# Autodesk Inventor assembly: Blesson Thomas_9005538_Final
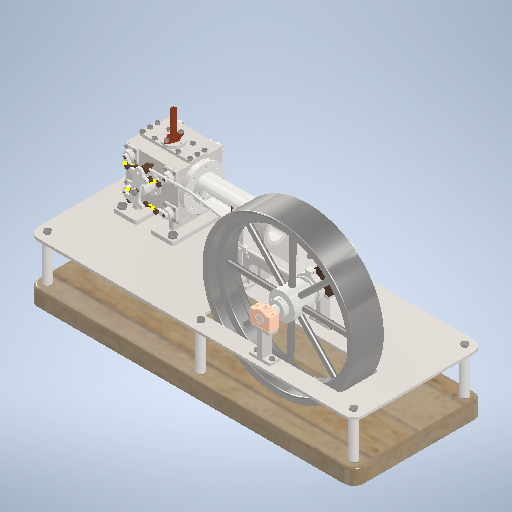
[picture p0: Inventor's stored thumbnail of the model, 512x512]
Saved by Autodesk Inventor 2025.2 (Build 292293000, 293)
## iProperties
Created: 2025-08-11
Part Number: Blesson Thomas_9005538_Final
Document SubType Name: Assembly
Designer: bless
Author: bless
## Documents named in this file (57)
- C:\Users\bless\OneDrive - Conestoga College\Documents\Inventor\pipe and flange\Blesson Thomas_9005538_Final\Blesson Thomas_9005538_Final.iam
- C:\Users\bless\OneDrive - Conestoga College\Documents\Inventor\pipe and flange\Blesson Thomas_9005538_Final\35 - Wooden Base.ipt
- C:\Users\bless\OneDrive - Conestoga College\Documents\Inventor\pipe and flange\Blesson Thomas_9005538_Final\34 - Base Pillar.ipt
- C:\Users\bless\OneDrive - Conestoga College\Documents\Inventor\Content Center Files\R2025\en-US\AS 1237 (2.1)\AS 1237 - 5.ipt
- C:\Users\bless\OneDrive - Conestoga College\Documents\Inventor\pipe and flange\Blesson Thomas_9005538_Final\01 - Base Plate\01 - Base Plate\01 - Base Plate.ipt
- C:\Users\bless\OneDrive - Conestoga College\Documents\Inventor\Content Center Files\R2025\en-US\AS 1110\AS 1110 - M4 x 40.ipt
- C:\Users\bless\OneDrive - Conestoga College\Documents\Inventor\pipe and flange\Blesson Thomas_9005538_Final\03 - Cylinder Foot\03 - Cylinder Foot\03 - Cylinder Foot.ipt
- C:\Users\bless\OneDrive - Conestoga College\Documents\Inventor\Content Center Files\R2025\en-US\AS 1110\AS 1110 - M5 x 12.ipt
- C:\Users\bless\OneDrive - Conestoga College\Documents\Inventor\pipe and flange\Blesson Thomas_9005538_Final\04A - Guide Support 1\04A - Guide Support 1\04A - Guide Support 1.ipt
- C:\Users\bless\OneDrive - Conestoga College\Documents\Inventor\Content Center Files\R2025\en-US\AS 1110\AS 1110 - M2.5 x 8.ipt
- C:\Users\bless\OneDrive - Conestoga College\Documents\Inventor\pipe and flange\Blesson Thomas_9005538_Final\04B - Guide Support 2\04B - Guide Support 2\04B - Guide Support 2.ipt
- C:\Users\bless\OneDrive - Conestoga College\Documents\Inventor\Content Center Files\R2025\en-US\AS 1110\AS 1110 - M2.5 x 12.ipt
- C:\Users\bless\OneDrive - Conestoga College\Documents\Inventor\pipe and flange\Blesson Thomas_9005538_Final\06 - Cylinder\06 - Cylinder\06 - Cylinder.ipt
- C:\Users\bless\OneDrive - Conestoga College\Documents\Inventor\pipe and flange\Blesson Thomas_9005538_Final\09 - Valve Chest Cover Plate\09 - Valve Chest Cover Plate\09 - Valve Chest Cover Plate.ipt
- C:\Users\bless\OneDrive - Conestoga College\Documents\Inventor\Content Center Files\R2025\en-US\AS 1110\AS 1110 - M2.5 x 6.ipt
- C:\Users\bless\OneDrive - Conestoga College\Documents\Inventor\pipe and flange\Blesson Thomas_9005538_Final\36 - Inlet Outlet Steam Pipe.ipt
- C:\Users\bless\OneDrive - Conestoga College\Documents\Inventor\pipe and flange\Blesson Thomas_9005538_Final\12B VALVE BONNET.ipt
- C:\Users\bless\OneDrive - Conestoga College\Documents\Inventor\Content Center Files\R2025\en-US\AS 1110\AS 1110 - M1.6 x 6.ipt
- C:\Users\bless\OneDrive - Conestoga College\Documents\Inventor\pipe and flange\Blesson Thomas_9005538_Final\07 CYLINDER FRONT COVER.ipt
- C:\Users\bless\OneDrive - Conestoga College\Documents\Inventor\pipe and flange\Blesson Thomas_9005538_Final\08 CYLINDER REAR COVER.ipt
- C:\Users\bless\OneDrive - Conestoga College\Documents\Inventor\pipe and flange\Blesson Thomas_9005538_Final\13A FLYWHEEL HUB.ipt
- C:\Users\bless\OneDrive - Conestoga College\Documents\Inventor\pipe and flange\Blesson Thomas_9005538_Final\Flywheel inner ring.ipt
- C:\Users\bless\OneDrive - Conestoga College\Documents\Inventor\pipe and flange\Blesson Thomas_9005538_Final\Flywheel outer rim.ipt
- C:\Users\bless\OneDrive - Conestoga College\Documents\Inventor\pipe and flange\Blesson Thomas_9005538_Final\Flywheel Spoke.ipt
- C:\Users\bless\OneDrive - Conestoga College\Documents\Inventor\pipe and flange\Blesson Thomas_9005538_Final\02 - Outrigger Bearing Pedestal\02 - Outrigger Bearing Pedestal\02 - Outrigger Bearing Pedestal.ipt
- C:\Users\bless\OneDrive - Conestoga College\Documents\Inventor\pipe and flange\Blesson Thomas_9005538_Final\05 Crankbearing.ipt
- C:\Users\bless\OneDrive - Conestoga College\Documents\Inventor\pipe and flange\Blesson Thomas_9005538_Final\02 - Outrigger Bearing Pedestal\05 - Crankshaft Bearing\05 - Crankshaft Bearing.ipt
- C:\Users\bless\OneDrive - Conestoga College\Documents\Inventor\pipe and flange\Blesson Thomas_9005538_Final\Crankshaft.ipt
- C:\Users\bless\OneDrive - Conestoga College\Documents\Inventor\pipe and flange\Blesson Thomas_9005538_Final\28 - Eccentric  Sheav.ipt
- C:\Users\bless\OneDrive - Conestoga College\Documents\Inventor\pipe and flange\Blesson Thomas_9005538_Final\29 - Sheave Strap 2.ipt
- C:\Users\bless\OneDrive - Conestoga College\Documents\Inventor\pipe and flange\Blesson Thomas_9005538_Final\29 - Sheave Strap 1.ipt
- C:\Users\bless\OneDrive - Conestoga College\Documents\Inventor\pipe and flange\Blesson Thomas_9005538_Final\30 - Eccentric Rod 1.ipt
- C:\Users\bless\OneDrive - Conestoga College\Documents\Inventor\pipe and flange\Blesson Thomas_9005538_Final\30 - Eccentric Rod 2.ipt
- C:\Users\bless\OneDrive - Conestoga College\Documents\Inventor\pipe and flange\Blesson Thomas_9005538_Final\31 - Lever.ipt
- C:\Users\bless\OneDrive - Conestoga College\Documents\Inventor\pipe and flange\Blesson Thomas_9005538_Final\32 - Eccentric Disk Rod.ipt
- C:\Users\bless\OneDrive - Conestoga College\Documents\Inventor\pipe and flange\Blesson Thomas_9005538_Final\22 - Valve Disc Hub.ipt
- C:\Users\bless\OneDrive - Conestoga College\Documents\Inventor\pipe and flange\Blesson Thomas_9005538_Final\33 - Eccentric Swivel Screw.ipt
- C:\Users\bless\OneDrive - Conestoga College\Documents\Inventor\pipe and flange\Blesson Thomas_9005538_Final\24 - Valve Disc Spindle.ipt
- C:\Users\bless\OneDrive - Conestoga College\Documents\Inventor\pipe and flange\Blesson Thomas_9005538_Final\23 - Valve Disc.ipt
- C:\Users\bless\OneDrive - Conestoga College\Documents\Inventor\Content Center Files\R2025\en-US\ANSI B18.2.4.2M\ANSI B18.2.4.2M - M3x0.5 - 5.5.ipt
- C:\Users\bless\OneDrive - Conestoga College\Documents\Inventor\pipe and flange\Blesson Thomas_9005538_Final\27 - Valve Level.ipt
- C:\Users\bless\OneDrive - Conestoga College\Documents\Inventor\pipe and flange\Blesson Thomas_9005538_Final\11 CROSSHEAD GUIDE.ipt
- C:\Users\bless\OneDrive - Conestoga College\Documents\Inventor\pipe and flange\Blesson Thomas_9005538_Final\25 - Disc Arm 1.ipt
- C:\Users\bless\OneDrive - Conestoga College\Documents\Inventor\pipe and flange\Blesson Thomas_9005538_Final\25 - Disc Arm 2.ipt
- C:\Users\bless\OneDrive - Conestoga College\Documents\Inventor\pipe and flange\Blesson Thomas_9005538_Final\26B - Valve spindle.ipt
- C:\Users\bless\OneDrive - Conestoga College\Documents\Inventor\pipe and flange\Blesson Thomas_9005538_Final\26A - Valve.ipt
- C:\Users\bless\OneDrive - Conestoga College\Documents\Inventor\pipe and flange\Blesson Thomas_9005538_Final\10a GLAND NUT.ipt
- C:\Users\bless\OneDrive - Conestoga College\Documents\Inventor\pipe and flange\Blesson Thomas_9005538_Final\10B - Gland Nut Seal\10B - Gland Nut Seal\10B - Gland Nut Seal.ipt
- C:\Users\bless\OneDrive - Conestoga College\Documents\Inventor\pipe and flange\Blesson Thomas_9005538_Final\16C - Con Head Crosshead.ipt
- C:\Users\bless\OneDrive - Conestoga College\Documents\Inventor\pipe and flange\Blesson Thomas_9005538_Final\19 - Crosshead.ipt
- C:\Users\bless\OneDrive - Conestoga College\Documents\Inventor\pipe and flange\Blesson Thomas_9005538_Final\18 - Piston Rod.ipt
- C:\Users\bless\OneDrive - Conestoga College\Documents\Inventor\pipe and flange\Blesson Thomas_9005538_Final\21 - Piston Ring.ipt
- C:\Users\bless\OneDrive - Conestoga College\Documents\Inventor\pipe and flange\Blesson Thomas_9005538_Final\20 - Piston.ipt
- C:\Users\bless\OneDrive - Conestoga College\Documents\Inventor\pipe and flange\Blesson Thomas_9005538_Final\16B2 - Con Head Big End.ipt
- C:\Users\bless\OneDrive - Conestoga College\Documents\Inventor\pipe and flange\Blesson Thomas_9005538_Final\16A - Con Rod.ipt
- C:\Users\bless\OneDrive - Conestoga College\Documents\Inventor\pipe and flange\Blesson Thomas_9005538_Final\17B - Crosshead Pin2.ipt
- C:\Users\bless\OneDrive - Conestoga College\Documents\Inventor\pipe and flange\Blesson Thomas_9005538_Final\Crankpin.ipt
## Components (176 placed, 56 different names)
1. 35 - Wooden Base:1 — Insert:1, Insert:2, Insert:3, Insert:4, Insert:5, Insert:6
2. 34 - Base Pillar:1 — Rigid:2
3. 34 - Base Pillar:2 — Rigid:4
4. 34 - Base Pillar:3 — Rigid:6, Cylindrical:1
5. 34 - Base Pillar:4 — Rigid:1, Rigid:7
6. 34 - Base Pillar:5 — Rigid:3
7. 34 - Base Pillar:6 — Rigid:5
8. AS 1237 (2.1) 5:1 — Insert:1, Rigid:1
9. AS 1237 (2.1) 5:2 — Insert:2, Rigid:2
10. AS 1237 (2.1) 5:3 — Insert:3, Rigid:4
11. AS 1237 (2.1) 5:4 — Insert:4, Rigid:5
12. AS 1237 (2.1) 5:5 — Insert:5, Rigid:6
13. AS 1237 (2.1) 5:6 — Insert:6, Rigid:3
14. 01 - Base Plate:1 — Rigid:7, Insert:7, Insert:8, Insert:9, Insert:10, Insert:11, Insert:12, Rotational:1, Cylindrical:2, Rotational:2, Cylindrical:3, Rotational:3, Cylindrical:4, Cylindrical:5, Cylindrical:6, Cylindrical:14, Cylindrical:44, Mate:27, Cylindrical:49
15. AS 1110 - Metric M4 x 40:1 — Insert:7
16. AS 1110 - Metric M4 x 40:2 — Insert:8
17. AS 1110 - Metric M4 x 40:3 — Insert:9
18. AS 1110 - Metric M4 x 40:4 — Insert:10
19. AS 1110 - Metric M4 x 40:5 — Insert:11
20. AS 1110 - Metric M4 x 40:6 — Insert:12, Cylindrical:1
21. 03 - Cylinder Foot:1 — Rotational:1, Insert:13, Insert:14
22. 03 - Cylinder Foot:2 — Rotational:2, Insert:15, Insert:16, Angle:1, Mate:7
23. AS 1110 - Metric M5 x 12:1 — Insert:13
24. AS 1110 - Metric M5 x 12:2 — Insert:14, Cylindrical:2
25. AS 1110 - Metric M5 x 12:3 — Insert:15
26. AS 1110 - Metric M5 x 12:4 — Insert:16, Cylindrical:3
27. 04A - Guide Support 1:1 — Insert:17, Insert:18, Rotational:3, Mate:1, Cylindrical:70
28. AS 1110 - Metric M2.5 x 8:1 — Insert:17
29. AS 1110 - Metric M2.5 x 8:2 — Insert:18, Cylindrical:4
30. 04B - Guide Support 2:1 — Mate:1, Insert:19, Insert:20, Cylindrical:45, Mate:28, Flush:3, Cylindrical:60
31. AS 1110 - Metric M2.5 x 12:1 — Insert:19, Cylindrical:5
32. AS 1110 - Metric M2.5 x 12:2 — Insert:20, Cylindrical:6
33. 06 - Cylinder:1 — Cylindrical:7, Mate:2, Cylindrical:13, Cylindrical:15, Cylindrical:16, Cylindrical:17, Mate:6, Mate:7, Cylindrical:18, Cylindrical:19, Mate:8, Cylindrical:20, Cylindrical:21, Mate:9, Cylindrical:22, Cylindrical:23, Mate:10, Cylindrical:24, Cylindrical:25, Mate:11, Cylindrical:26, Cylindrical:27, Mate:12, Mate:13, Cylindrical:28, Cylindrical:29, Mate:14, Cylindrical:30, Cylindrical:31, Cylindrical:32, Cylindrical:33, Mate:16, Mate:17, Cylindrical:61, Mate:40
34. 09 - Valve Chest Cover Plate:1 — Insert:21, Insert:22, Insert:23, Insert:24, Insert:25, Insert:26, Insert:27, Insert:28, Insert:29, Insert:30, Mate:2, Cylindrical:11, Cylindrical:12, Mate:5
35. 09 - Valve Chest Cover Plate:2 — Insert:32, Insert:33, Insert:34, Insert:35, Insert:36, Insert:37, Insert:38, Insert:39, Insert:40, Cylindrical:9, Cylindrical:10, Mate:4, Mate:6, Angle:1
36. AS 1110 - Metric M2.5 x 6:1 — Insert:21
37. AS 1110 - Metric M2.5 x 6:2 — Insert:22, Cylindrical:7
38. AS 1110 - Metric M2.5 x 6:3 — Insert:23
39. AS 1110 - Metric M2.5 x 6:4 — Insert:24
40. AS 1110 - Metric M2.5 x 6:5 — Insert:25
41. AS 1110 - Metric M2.5 x 6:6 — Insert:26, Cylindrical:13
42. AS 1110 - Metric M2.5 x 6:7 — Insert:27
43. AS 1110 - Metric M2.5 x 6:8 — Insert:28
44. AS 1110 - Metric M2.5 x 6:9 — Insert:29
45. AS 1110 - Metric M2.5 x 6:10 — Insert:30
46. AS 1110 - Metric M2.5 x 6:12 — Insert:32
47. AS 1110 - Metric M2.5 x 6:13 — Insert:33, Cylindrical:17
48. AS 1110 - Metric M2.5 x 6:14 — Insert:34
49. AS 1110 - Metric M2.5 x 6:15 — Insert:35
50. AS 1110 - Metric M2.5 x 6:16 — Insert:36, Cylindrical:15
51. AS 1110 - Metric M2.5 x 6:17 — Insert:37
52. AS 1110 - Metric M2.5 x 6:18 — Insert:38
53. AS 1110 - Metric M2.5 x 6:19 — Insert:39, Cylindrical:16
54. AS 1110 - Metric M2.5 x 6:20 — Insert:40
55. 36 - Inlet Outlet Steam Pipe:1 — Insert:43, Insert:44, Mate:5
56. 36 - Inlet Outlet Steam Pipe:2 — Insert:41, Insert:42, Mate:4, Cylindrical:14
57. AS 1110 - Metric M2.5 x 6:21 — Insert:41, Cylindrical:9
58. AS 1110 - Metric M2.5 x 6:22 — Insert:42, Cylindrical:10
59. AS 1110 - Metric M2.5 x 6:23 — Insert:43, Cylindrical:11
60. AS 1110 - Metric M2.5 x 6:24 — Insert:44, Cylindrical:12
61. 12B VALVE BONNET:1 — Insert:61, Insert:62, Insert:63, Insert:64, Mate:9, Cylindrical:66, Mate:46
62. 12B VALVE BONNET:2 — Insert:65, Insert:66, Insert:67, Insert:68, Mate:11, Cylindrical:67, Mate:47
63. 12B VALVE BONNET:3 — Insert:73, Insert:74, Insert:75, Insert:76, Mate:8, Cylindrical:65, Mate:45
64. 12B VALVE BONNET:4 — Insert:69, Insert:70, Insert:71, Insert:72, Mate:10, Cylindrical:68, Mate:48
65. 12B VALVE BONNET:5 — Insert:57, Insert:58, Insert:59, Insert:60, Mate:13, Cylindrical:28
66. 12B VALVE BONNET:6 — Insert:53, Insert:54, Insert:55, Insert:56, Flush:1
67. 12B VALVE BONNET:7 — Insert:45, Insert:46, Insert:47, Insert:48, Cylindrical:29, Mate:14, Flush:1
68. 12B VALVE BONNET:8 — Insert:49, Insert:50, Insert:51, Insert:52, Mate:12
69. AS 1110 - Metric M1.6 x 6:1 — Insert:45
70. AS 1110 - Metric M1.6 x 6:2 — Insert:46
71. AS 1110 - Metric M1.6 x 6:3 — Insert:47
72. AS 1110 - Metric M1.6 x 6:4 — Insert:48, Cylindrical:30
73. AS 1110 - Metric M1.6 x 6:5 — Insert:49, Cylindrical:27
74. AS 1110 - Metric M1.6 x 6:6 — Insert:50
75. AS 1110 - Metric M1.6 x 6:7 — Insert:51, Cylindrical:26
76. AS 1110 - Metric M1.6 x 6:8 — Insert:52
77. AS 1110 - Metric M1.6 x 6:9 — Insert:53, Cylindrical:32
78. AS 1110 - Metric M1.6 x 6:10 — Insert:54, Cylindrical:33
79. AS 1110 - Metric M1.6 x 6:11 — Insert:55
80. AS 1110 - Metric M1.6 x 6:12 — Insert:56
81. AS 1110 - Metric M1.6 x 6:13 — Insert:57
82. AS 1110 - Metric M1.6 x 6:14 — Insert:58
83. AS 1110 - Metric M1.6 x 6:15 — Insert:59
84. AS 1110 - Metric M1.6 x 6:16 — Insert:60, Cylindrical:31
85. AS 1110 - Metric M1.6 x 6:17 — Insert:61
86. AS 1110 - Metric M1.6 x 6:18 — Insert:62, Cylindrical:21
87. AS 1110 - Metric M1.6 x 6:19 — Insert:63, Cylindrical:20
88. AS 1110 - Metric M1.6 x 6:20 — Insert:64
89. AS 1110 - Metric M1.6 x 6:21 — Insert:65
90. AS 1110 - Metric M1.6 x 6:22 — Insert:66, Cylindrical:25
91. AS 1110 - Metric M1.6 x 6:23 — Insert:67, Cylindrical:24
92. AS 1110 - Metric M1.6 x 6:24 — Insert:68
93. AS 1110 - Metric M1.6 x 6:25 — Insert:69, Cylindrical:23
94. AS 1110 - Metric M1.6 x 6:26 — Insert:70, Cylindrical:22
95. AS 1110 - Metric M1.6 x 6:27 — Insert:71
96. AS 1110 - Metric M1.6 x 6:28 — Insert:72
97. AS 1110 - Metric M1.6 x 6:29 — Insert:73, Cylindrical:18
98. AS 1110 - Metric M1.6 x 6:30 — Insert:74, Cylindrical:19
99. AS 1110 - Metric M1.6 x 6:31 — Insert:75
100. AS 1110 - Metric M1.6 x 6:32 — Insert:76
101. 07 CYLINDER FRONT COVER:1 — Insert:77, Insert:78, Insert:79, Insert:80, Insert:81, Insert:82, Insert:83, Insert:84, Mate:16
102. AS 1110 - Metric M2.5 x 6:25 — Insert:77
103. AS 1110 - Metric M2.5 x 6:26 — Insert:78
104. AS 1110 - Metric M2.5 x 6:27 — Insert:79
105. AS 1110 - Metric M2.5 x 6:28 — Insert:80
106. AS 1110 - Metric M2.5 x 6:29 — Insert:81
107. AS 1110 - Metric M2.5 x 6:30 — Insert:82
108. AS 1110 - Metric M2.5 x 6:31 — Insert:83
109. AS 1110 - Metric M2.5 x 6:32 — Insert:84
110. 08 CYLINDER REAR COVER:1 — Mate:17, Cylindrical:69, Mate:71, Mate:74
111. 13A FLYWHEEL HUB:1 — Cylindrical:34, Cylindrical:35, Cylindrical:36, Cylindrical:37, Mate:15, Mate:18, Mate:19, Mate:20, Cylindrical:38, Mate:21, Cylindrical:39, Cylindrical:40, Cylindrical:41, Mate:22, Mate:23, Mate:24, Cylindrical:51, Cylindrical:52, Cylindrical:54
112. Flywheel inner ring:1 — Cylindrical:42, Cylindrical:43, Mate:25, Insert:95
113. Flywheel outer rim:1 — Mate:25, Insert:95
114. Flywheel Spoke:1 — Cylindrical:34, Mate:18
115. Flywheel Spoke:2 — Cylindrical:39, Mate:24
116. Flywheel Spoke:3 — Cylindrical:38, Mate:21
117. Flywheel Spoke:4 — Cylindrical:35, Mate:15
118. Flywheel Spoke:5 — Cylindrical:40, Mate:22, Cylindrical:42
119. Flywheel Spoke:6 — Cylindrical:41, Mate:23, Cylindrical:43
120. Flywheel Spoke:7 — Cylindrical:37, Mate:20
121. Flywheel Spoke:8 — Cylindrical:36, Mate:19
122. 02 - Outrigger Bearing Pedestal:2 — Insert:93, Insert:94, Mate:26, Mate:27, Flush:2, Mate:29, Flush:4
123. AS 1110 - Metric M2.5 x 6:41 — Insert:93, Cylindrical:44
124. AS 1110 - Metric M2.5 x 6:42 — Insert:94, Cylindrical:49
125. 05 Crankbearing:1 — Cylindrical:45, Mate:28, Flush:3
126. 05 - Crankshaft Bearing:1 — Mate:26, Flush:2, Mate:29, Flush:4, Flush:5, Cylindrical:50, Cylindrical:51
127. Crankshaft:1 — Flush:5, Cylindrical:50, Cylindrical:52, Mate:31, Cylindrical:96
128. 28 - Eccentric  Sheav:1 — Mate:31, Mate:33, Flush:7, Cylindrical:54, Mate:35
129. 29 - Sheave Strap 2:1 — Cylindrical:53, Mate:32, Mate:34, Flush:6, Flush:7
130. 29 - Sheave Strap 1:1 — Cylindrical:53, Mate:32, Mate:33, Mate:34, Flush:6, Cylindrical:55
131. 30 - Eccentric Rod 1:1 — Cylindrical:55, Mate:35, Cylindrical:56, Mate:36
132. 30 - Eccentric Rod 2:1 — Cylindrical:56, Mate:36, Cylindrical:57, Mate:37
133. 31 - Lever:1 — Cylindrical:57, Mate:37, Cylindrical:59, Mate:39, Cylindrical:60
134. 32 - Eccentric Disk Rod:1 — Cylindrical:58, Mate:38, Cylindrical:62
135. 30 - Eccentric Rod 2:2 — Cylindrical:58, Mate:38, Cylindrical:59, Mate:39
136. 22 - Valve Disc Hub:2 — Cylindrical:61, Mate:40, Cylindrical:63, Flush:8
137. 33 - Eccentric Swivel Screw:1 — Cylindrical:62, Cylindrical:64
138. 24 - Valve Disc Spindle:1 — Cylindrical:63, Flush:8, Mate:41, Mate:42, Flush:9, Mate:43, Mate:44
139. 23 - Valve Disc:1 — Mate:41, Mate:42, Cylindrical:64, Flush:9, Cylindrical:75, Cylindrical:76, Cylindrical:77, Cylindrical:78
140. ANSI B18.2.4.2M M3x0.5:1 — Mate:43, Mate:44
141. 27 - Valve Level:1 — Cylindrical:65, Mate:45, Cylindrical:71, Mate:58, Cylindrical:84
142. 27 - Valve Level:2 — Cylindrical:66, Mate:46, Cylindrical:72, Mate:59, Cylindrical:85
143. 27 - Valve Level:3 — Cylindrical:67, Mate:47, Cylindrical:74, Mate:60, Cylindrical:86
144. 27 - Valve Level:4 — Cylindrical:68, Mate:48, Cylindrical:73, Mate:61, Cylindrical:83
145. 11 CROSSHEAD GUIDE:1 — Cylindrical:69, Cylindrical:70, Cylindrical:91, Mate:74
146. 25 - Disc Arm 1:1 — Mate:56, Cylindrical:76
147. 25 - Disc Arm 1:2 — Mate:54, Cylindrical:73, Mate:61
148. 25 - Disc Arm 1:3 — Mate:52, Cylindrical:78
149. 25 - Disc Arm 1:4 — Mate:49, Mate:50, Mate:58, Cylindrical:75
150. 25 - Disc Arm 1:5 — Mate:51, Cylindrical:71
151. 25 - Disc Arm 1:6 — Mate:53, Cylindrical:74, Mate:60
152. 25 - Disc Arm 1:7 — Mate:55, Cylindrical:77
153. 25 - Disc Arm 1:8 — Mate:57, Cylindrical:72, Mate:59
154. 25 - Disc Arm 2:1 — Mate:49, Mate:50, Mate:51
155. 25 - Disc Arm 2:2 — Mate:52, Mate:53
156. 25 - Disc Arm 2:3 — Mate:54, Mate:55
157. 25 - Disc Arm 2:4 — Mate:56, Mate:57
158. 26B - Valve spindle:1 — Mate:62, Cylindrical:79, Mate:63, Cylindrical:83
159. 26A - Valve:1 — Mate:62, Cylindrical:79, Mate:63
160. 26B - Valve spindle:2 — Cylindrical:84
161. 26A - Valve:2
162. 26B - Valve spindle:3 — Cylindrical:85
163. 26A - Valve:3
164. 26B - Valve spindle:4 — Cylindrical:86
165. 26A - Valve:4
166. 10a GLAND NUT:1 — Cylindrical:87, Mate:70
167. 10B - Gland Nut Seal:1 — Cylindrical:87, Mate:70, Mate:71
168. 16C - Con Head Crosshead:1 — Mate:76, Cylindrical:92, Mate:77, Cylindrical:94, Mate:78
169. 19 - Crosshead:1 — Cylindrical:88, Mate:72, Cylindrical:93, Mate:78
170. 18 - Piston Rod:1 — Cylindrical:88, Mate:72, Cylindrical:90, Flush:10
171. 21 - Piston Ring:1 — Cylindrical:89, Mate:73
172. 20 - Piston:1 — Cylindrical:89, Mate:73, Cylindrical:90, Flush:10, Cylindrical:91
173. 16B2 - Con Head Big End:1 — Mate:75, Cylindrical:95, Cylindrical:96, Cylindrical:97
174. 16A - Con Rod:1 — Mate:75, Mate:76, Cylindrical:94, Cylindrical:95
175. 17B - Crosshead Pin2:1 — Cylindrical:92, Mate:77, Cylindrical:93
176. Crankpin:1 — Cylindrical:97
## Relationships (276: CylindricalJoint 93, Insert 86, Mate 76, Flush 10, WeldJoint 7, RevoluteJoint 3, Angle 1)
- Insert:1: 35 - Wooden Base:1 ↔ AS 1237 (2.1) 5:1
- Insert:2: 35 - Wooden Base:1 ↔ AS 1237 (2.1) 5:2
- Insert:3: 35 - Wooden Base:1 ↔ AS 1237 (2.1) 5:3
- Insert:4: 35 - Wooden Base:1 ↔ AS 1237 (2.1) 5:4
- Insert:5: 35 - Wooden Base:1 ↔ AS 1237 (2.1) 5:5
- Insert:6: 35 - Wooden Base:1 ↔ AS 1237 (2.1) 5:6
- Rigid:1 [WeldJoint]: 34 - Base Pillar:4 ↔ AS 1237 (2.1) 5:1
- Rigid:2 [WeldJoint]: 34 - Base Pillar:1 ↔ AS 1237 (2.1) 5:2
- Rigid:3 [WeldJoint]: 34 - Base Pillar:5 ↔ AS 1237 (2.1) 5:6
- Rigid:4 [WeldJoint]: 34 - Base Pillar:2 ↔ AS 1237 (2.1) 5:3
- Rigid:5 [WeldJoint]: 34 - Base Pillar:6 ↔ AS 1237 (2.1) 5:4
- Rigid:6 [WeldJoint]: 34 - Base Pillar:3 ↔ AS 1237 (2.1) 5:5
- Rigid:7 [WeldJoint]: 34 - Base Pillar:4 ↔ 01 - Base Plate:1
- Insert:7: 01 - Base Plate:1 ↔ AS 1110 - Metric M4 x 40:1
- Insert:8: 01 - Base Plate:1 ↔ AS 1110 - Metric M4 x 40:2
- Insert:9: 01 - Base Plate:1 ↔ AS 1110 - Metric M4 x 40:3
- Insert:10: 01 - Base Plate:1 ↔ AS 1110 - Metric M4 x 40:4
- Insert:11: 01 - Base Plate:1 ↔ AS 1110 - Metric M4 x 40:5
- Insert:12: 01 - Base Plate:1 ↔ AS 1110 - Metric M4 x 40:6
- Rotational:1 [RevoluteJoint]: 01 - Base Plate:1 ↔ 03 - Cylinder Foot:1
- Cylindrical:1: 34 - Base Pillar:3 ↔ AS 1110 - Metric M4 x 40:6
- Insert:13: 03 - Cylinder Foot:1 ↔ AS 1110 - Metric M5 x 12:1
- Insert:14: 03 - Cylinder Foot:1 ↔ AS 1110 - Metric M5 x 12:2
- Cylindrical:2: 01 - Base Plate:1 ↔ AS 1110 - Metric M5 x 12:2
- Rotational:2 [RevoluteJoint]: 01 - Base Plate:1 ↔ 03 - Cylinder Foot:2
- Insert:15: 03 - Cylinder Foot:2 ↔ AS 1110 - Metric M5 x 12:3
- Insert:16: 03 - Cylinder Foot:2 ↔ AS 1110 - Metric M5 x 12:4
- Cylindrical:3: 01 - Base Plate:1 ↔ AS 1110 - Metric M5 x 12:4
- Insert:17: 04A - Guide Support 1:1 ↔ AS 1110 - Metric M2.5 x 8:1
- Insert:18: 04A - Guide Support 1:1 ↔ AS 1110 - Metric M2.5 x 8:2
- Rotational:3 [RevoluteJoint]: 01 - Base Plate:1 ↔ 04A - Guide Support 1:1
- Cylindrical:4: 01 - Base Plate:1 ↔ AS 1110 - Metric M2.5 x 8:2
- Mate:1: 04A - Guide Support 1:1 ↔ 04B - Guide Support 2:1
- Insert:19: 04B - Guide Support 2:1 ↔ AS 1110 - Metric M2.5 x 12:1
- Insert:20: 04B - Guide Support 2:1 ↔ AS 1110 - Metric M2.5 x 12:2
- Cylindrical:5: 01 - Base Plate:1 ↔ AS 1110 - Metric M2.5 x 12:1
- Cylindrical:6: 01 - Base Plate:1 ↔ AS 1110 - Metric M2.5 x 12:2
- Insert:21: 09 - Valve Chest Cover Plate:1 ↔ AS 1110 - Metric M2.5 x 6:1
- Insert:22: 09 - Valve Chest Cover Plate:1 ↔ AS 1110 - Metric M2.5 x 6:2
- Insert:23: 09 - Valve Chest Cover Plate:1 ↔ AS 1110 - Metric M2.5 x 6:3
- Insert:24: 09 - Valve Chest Cover Plate:1 ↔ AS 1110 - Metric M2.5 x 6:4
- Insert:25: 09 - Valve Chest Cover Plate:1 ↔ AS 1110 - Metric M2.5 x 6:5
- Insert:26: 09 - Valve Chest Cover Plate:1 ↔ AS 1110 - Metric M2.5 x 6:6
- Insert:27: 09 - Valve Chest Cover Plate:1 ↔ AS 1110 - Metric M2.5 x 6:7
- Insert:28: 09 - Valve Chest Cover Plate:1 ↔ AS 1110 - Metric M2.5 x 6:8
- Insert:29: 09 - Valve Chest Cover Plate:1 ↔ AS 1110 - Metric M2.5 x 6:9
- Insert:30: 09 - Valve Chest Cover Plate:1 ↔ AS 1110 - Metric M2.5 x 6:10
- Cylindrical:7: 06 - Cylinder:1 ↔ AS 1110 - Metric M2.5 x 6:2
- Mate:2: 06 - Cylinder:1 ↔ 09 - Valve Chest Cover Plate:1
- Insert:32: 09 - Valve Chest Cover Plate:2 ↔ AS 1110 - Metric M2.5 x 6:12
- Insert:33: 09 - Valve Chest Cover Plate:2 ↔ AS 1110 - Metric M2.5 x 6:13
- Insert:34: 09 - Valve Chest Cover Plate:2 ↔ AS 1110 - Metric M2.5 x 6:14
- Insert:35: 09 - Valve Chest Cover Plate:2 ↔ AS 1110 - Metric M2.5 x 6:15
- Insert:36: 09 - Valve Chest Cover Plate:2 ↔ AS 1110 - Metric M2.5 x 6:16
- Insert:37: 09 - Valve Chest Cover Plate:2 ↔ AS 1110 - Metric M2.5 x 6:17
- Insert:38: 09 - Valve Chest Cover Plate:2 ↔ AS 1110 - Metric M2.5 x 6:18
- Insert:39: 09 - Valve Chest Cover Plate:2 ↔ AS 1110 - Metric M2.5 x 6:19
- Insert:40: 09 - Valve Chest Cover Plate:2 ↔ AS 1110 - Metric M2.5 x 6:20
- Insert:41: 36 - Inlet Outlet Steam Pipe:2 ↔ AS 1110 - Metric M2.5 x 6:21
- Insert:42: 36 - Inlet Outlet Steam Pipe:2 ↔ AS 1110 - Metric M2.5 x 6:22
- Insert:43: 36 - Inlet Outlet Steam Pipe:1 ↔ AS 1110 - Metric M2.5 x 6:23
- Insert:44: 36 - Inlet Outlet Steam Pipe:1 ↔ AS 1110 - Metric M2.5 x 6:24
- Cylindrical:9: 09 - Valve Chest Cover Plate:2 ↔ AS 1110 - Metric M2.5 x 6:21
- Cylindrical:10: 09 - Valve Chest Cover Plate:2 ↔ AS 1110 - Metric M2.5 x 6:22
- Mate:4: 09 - Valve Chest Cover Plate:2 ↔ 36 - Inlet Outlet Steam Pipe:2
- Cylindrical:11: 09 - Valve Chest Cover Plate:1 ↔ AS 1110 - Metric M2.5 x 6:23
- Cylindrical:12: 09 - Valve Chest Cover Plate:1 ↔ AS 1110 - Metric M2.5 x 6:24
- Mate:5: 09 - Valve Chest Cover Plate:1 ↔ 36 - Inlet Outlet Steam Pipe:1
- Cylindrical:13: 06 - Cylinder:1 ↔ AS 1110 - Metric M2.5 x 6:6
- Cylindrical:14: 01 - Base Plate:1 ↔ 36 - Inlet Outlet Steam Pipe:2
- Cylindrical:15: 06 - Cylinder:1 ↔ AS 1110 - Metric M2.5 x 6:16
- Cylindrical:16: 06 - Cylinder:1 ↔ AS 1110 - Metric M2.5 x 6:19
- Cylindrical:17: 06 - Cylinder:1 ↔ AS 1110 - Metric M2.5 x 6:13
- Mate:6: 06 - Cylinder:1 ↔ 09 - Valve Chest Cover Plate:2
- Angle:1 (0 deg): 03 - Cylinder Foot:2 ↔ 09 - Valve Chest Cover Plate:2
- Mate:7: 03 - Cylinder Foot:2 ↔ 06 - Cylinder:1
- Insert:45: 12B VALVE BONNET:7 ↔ AS 1110 - Metric M1.6 x 6:1
- Insert:46: 12B VALVE BONNET:7 ↔ AS 1110 - Metric M1.6 x 6:2
- Insert:47: 12B VALVE BONNET:7 ↔ AS 1110 - Metric M1.6 x 6:3
- Insert:48: 12B VALVE BONNET:7 ↔ AS 1110 - Metric M1.6 x 6:4
- Insert:49: 12B VALVE BONNET:8 ↔ AS 1110 - Metric M1.6 x 6:5
- Insert:50: 12B VALVE BONNET:8 ↔ AS 1110 - Metric M1.6 x 6:6
- Insert:51: 12B VALVE BONNET:8 ↔ AS 1110 - Metric M1.6 x 6:7
- Insert:52: 12B VALVE BONNET:8 ↔ AS 1110 - Metric M1.6 x 6:8
- Insert:53: 12B VALVE BONNET:6 ↔ AS 1110 - Metric M1.6 x 6:9
- Insert:54: 12B VALVE BONNET:6 ↔ AS 1110 - Metric M1.6 x 6:10
- Insert:55: 12B VALVE BONNET:6 ↔ AS 1110 - Metric M1.6 x 6:11
- Insert:56: 12B VALVE BONNET:6 ↔ AS 1110 - Metric M1.6 x 6:12
- Insert:57: 12B VALVE BONNET:5 ↔ AS 1110 - Metric M1.6 x 6:13
- Insert:58: 12B VALVE BONNET:5 ↔ AS 1110 - Metric M1.6 x 6:14
- Insert:59: 12B VALVE BONNET:5 ↔ AS 1110 - Metric M1.6 x 6:15
- Insert:60: 12B VALVE BONNET:5 ↔ AS 1110 - Metric M1.6 x 6:16
- Insert:61: 12B VALVE BONNET:1 ↔ AS 1110 - Metric M1.6 x 6:17
- Insert:62: 12B VALVE BONNET:1 ↔ AS 1110 - Metric M1.6 x 6:18
- Insert:63: 12B VALVE BONNET:1 ↔ AS 1110 - Metric M1.6 x 6:19
- Insert:64: 12B VALVE BONNET:1 ↔ AS 1110 - Metric M1.6 x 6:20
- Insert:65: 12B VALVE BONNET:2 ↔ AS 1110 - Metric M1.6 x 6:21
- Insert:66: 12B VALVE BONNET:2 ↔ AS 1110 - Metric M1.6 x 6:22
- Insert:67: 12B VALVE BONNET:2 ↔ AS 1110 - Metric M1.6 x 6:23
- Insert:68: 12B VALVE BONNET:2 ↔ AS 1110 - Metric M1.6 x 6:24
- Insert:69: 12B VALVE BONNET:4 ↔ AS 1110 - Metric M1.6 x 6:25
- Insert:70: 12B VALVE BONNET:4 ↔ AS 1110 - Metric M1.6 x 6:26
- Insert:71: 12B VALVE BONNET:4 ↔ AS 1110 - Metric M1.6 x 6:27
- Insert:72: 12B VALVE BONNET:4 ↔ AS 1110 - Metric M1.6 x 6:28
- Insert:73: 12B VALVE BONNET:3 ↔ AS 1110 - Metric M1.6 x 6:29
- Insert:74: 12B VALVE BONNET:3 ↔ AS 1110 - Metric M1.6 x 6:30
- Insert:75: 12B VALVE BONNET:3 ↔ AS 1110 - Metric M1.6 x 6:31
- Insert:76: 12B VALVE BONNET:3 ↔ AS 1110 - Metric M1.6 x 6:32
- Cylindrical:18: 06 - Cylinder:1 ↔ AS 1110 - Metric M1.6 x 6:29
- Cylindrical:19: 06 - Cylinder:1 ↔ AS 1110 - Metric M1.6 x 6:30
- Mate:8: 06 - Cylinder:1 ↔ 12B VALVE BONNET:3
- Cylindrical:20: 06 - Cylinder:1 ↔ AS 1110 - Metric M1.6 x 6:19
- Cylindrical:21: 06 - Cylinder:1 ↔ AS 1110 - Metric M1.6 x 6:18
- Mate:9: 06 - Cylinder:1 ↔ 12B VALVE BONNET:1
- Cylindrical:22: 06 - Cylinder:1 ↔ AS 1110 - Metric M1.6 x 6:26
- Cylindrical:23: 06 - Cylinder:1 ↔ AS 1110 - Metric M1.6 x 6:25
- Mate:10: 06 - Cylinder:1 ↔ 12B VALVE BONNET:4
- Cylindrical:24: 06 - Cylinder:1 ↔ AS 1110 - Metric M1.6 x 6:23
- Cylindrical:25: 06 - Cylinder:1 ↔ AS 1110 - Metric M1.6 x 6:22
- Mate:11: 06 - Cylinder:1 ↔ 12B VALVE BONNET:2
- Cylindrical:26: 06 - Cylinder:1 ↔ AS 1110 - Metric M1.6 x 6:7
- Cylindrical:27: 06 - Cylinder:1 ↔ AS 1110 - Metric M1.6 x 6:5
- Mate:12: 06 - Cylinder:1 ↔ 12B VALVE BONNET:8
- Mate:13: 06 - Cylinder:1 ↔ 12B VALVE BONNET:5
- Cylindrical:28: 06 - Cylinder:1 ↔ 12B VALVE BONNET:5
- Cylindrical:29: 06 - Cylinder:1 ↔ 12B VALVE BONNET:7
- Mate:14: 06 - Cylinder:1 ↔ 12B VALVE BONNET:7
- Cylindrical:30: 06 - Cylinder:1 ↔ AS 1110 - Metric M1.6 x 6:4
- Cylindrical:31: 06 - Cylinder:1 ↔ AS 1110 - Metric M1.6 x 6:16
- Cylindrical:32: 06 - Cylinder:1 ↔ AS 1110 - Metric M1.6 x 6:9
- Cylindrical:33: 06 - Cylinder:1 ↔ AS 1110 - Metric M1.6 x 6:10
- Flush:1: 12B VALVE BONNET:6 ↔ 12B VALVE BONNET:7
- Insert:77: 07 CYLINDER FRONT COVER:1 ↔ AS 1110 - Metric M2.5 x 6:25
- Insert:78: 07 CYLINDER FRONT COVER:1 ↔ AS 1110 - Metric M2.5 x 6:26
- Insert:79: 07 CYLINDER FRONT COVER:1 ↔ AS 1110 - Metric M2.5 x 6:27
- Insert:80: 07 CYLINDER FRONT COVER:1 ↔ AS 1110 - Metric M2.5 x 6:28
- Insert:81: 07 CYLINDER FRONT COVER:1 ↔ AS 1110 - Metric M2.5 x 6:29
- Insert:82: 07 CYLINDER FRONT COVER:1 ↔ AS 1110 - Metric M2.5 x 6:30
- Insert:83: 07 CYLINDER FRONT COVER:1 ↔ AS 1110 - Metric M2.5 x 6:31
- Insert:84: 07 CYLINDER FRONT COVER:1 ↔ AS 1110 - Metric M2.5 x 6:32
- Cylindrical:34: 13A FLYWHEEL HUB:1 ↔ Flywheel Spoke:1
- Cylindrical:35: 13A FLYWHEEL HUB:1 ↔ Flywheel Spoke:4
- Cylindrical:36: 13A FLYWHEEL HUB:1 ↔ Flywheel Spoke:8
- Cylindrical:37: 13A FLYWHEEL HUB:1 ↔ Flywheel Spoke:7
- Mate:15: 13A FLYWHEEL HUB:1 ↔ Flywheel Spoke:4
- Mate:16: 06 - Cylinder:1 ↔ 07 CYLINDER FRONT COVER:1
- Mate:17: 06 - Cylinder:1 ↔ 08 CYLINDER REAR COVER:1
- Mate:18: 13A FLYWHEEL HUB:1 ↔ Flywheel Spoke:1
- Mate:19: 13A FLYWHEEL HUB:1 ↔ Flywheel Spoke:8
- Mate:20: 13A FLYWHEEL HUB:1 ↔ Flywheel Spoke:7
- Cylindrical:38: 13A FLYWHEEL HUB:1 ↔ Flywheel Spoke:3
- Mate:21: 13A FLYWHEEL HUB:1 ↔ Flywheel Spoke:3
- Cylindrical:39: 13A FLYWHEEL HUB:1 ↔ Flywheel Spoke:2
- Cylindrical:40: 13A FLYWHEEL HUB:1 ↔ Flywheel Spoke:5
- Cylindrical:41: 13A FLYWHEEL HUB:1 ↔ Flywheel Spoke:6
- Mate:22: 13A FLYWHEEL HUB:1 ↔ Flywheel Spoke:5
- Mate:23: 13A FLYWHEEL HUB:1 ↔ Flywheel Spoke:6
- Mate:24: 13A FLYWHEEL HUB:1 ↔ Flywheel Spoke:2
- Cylindrical:42: Flywheel inner ring:1 ↔ Flywheel Spoke:5
- Cylindrical:43: Flywheel inner ring:1 ↔ Flywheel Spoke:6
- Mate:25: Flywheel inner ring:1 ↔ Flywheel outer rim:1
- Insert:93: 02 - Outrigger Bearing Pedestal:2 ↔ AS 1110 - Metric M2.5 x 6:41
- Insert:94: 02 - Outrigger Bearing Pedestal:2 ↔ AS 1110 - Metric M2.5 x 6:42
- Cylindrical:44: 01 - Base Plate:1 ↔ AS 1110 - Metric M2.5 x 6:41
- Cylindrical:45: 04B - Guide Support 2:1 ↔ 05 Crankbearing:1
- Mate:26: 02 - Outrigger Bearing Pedestal:2 ↔ 05 - Crankshaft Bearing:1
- Mate:27: 01 - Base Plate:1 ↔ 02 - Outrigger Bearing Pedestal:2
- Flush:2: 02 - Outrigger Bearing Pedestal:2 ↔ 05 - Crankshaft Bearing:1
- Mate:28: 04B - Guide Support 2:1 ↔ 05 Crankbearing:1
- Flush:3: 04B - Guide Support 2:1 ↔ 05 Crankbearing:1
- Cylindrical:49: 01 - Base Plate:1 ↔ AS 1110 - Metric M2.5 x 6:42
- Mate:29: 02 - Outrigger Bearing Pedestal:2 ↔ 05 - Crankshaft Bearing:1
- Flush:4: 02 - Outrigger Bearing Pedestal:2 ↔ 05 - Crankshaft Bearing:1
- Insert:95 (8 mm): Flywheel inner ring:1 ↔ Flywheel outer rim:1
- Flush:5: 05 - Crankshaft Bearing:1 ↔ Crankshaft:1
- Cylindrical:50: 05 - Crankshaft Bearing:1 ↔ Crankshaft:1
- Cylindrical:51: 13A FLYWHEEL HUB:1 ↔ 05 - Crankshaft Bearing:1
- Cylindrical:52: 13A FLYWHEEL HUB:1 ↔ Crankshaft:1
- Mate:31 (18 mm): Crankshaft:1 ↔ 28 - Eccentric  Sheav:1
- Cylindrical:53: 29 - Sheave Strap 2:1 ↔ 29 - Sheave Strap 1:1
- Mate:32: 29 - Sheave Strap 2:1 ↔ 29 - Sheave Strap 1:1
- Mate:33: 28 - Eccentric  Sheav:1 ↔ 29 - Sheave Strap 1:1
- Mate:34: 29 - Sheave Strap 2:1 ↔ 29 - Sheave Strap 1:1
- Flush:6: 29 - Sheave Strap 2:1 ↔ 29 - Sheave Strap 1:1
- Flush:7: 28 - Eccentric  Sheav:1 ↔ 29 - Sheave Strap 2:1
- Cylindrical:54: 13A FLYWHEEL HUB:1 ↔ 28 - Eccentric  Sheav:1
- Cylindrical:55: 29 - Sheave Strap 1:1 ↔ 30 - Eccentric Rod 1:1
- Mate:35: 28 - Eccentric  Sheav:1 ↔ 30 - Eccentric Rod 1:1
- Cylindrical:56: 30 - Eccentric Rod 1:1 ↔ 30 - Eccentric Rod 2:1
- Mate:36: 30 - Eccentric Rod 1:1 ↔ 30 - Eccentric Rod 2:1
- Cylindrical:57: 30 - Eccentric Rod 2:1 ↔ 31 - Lever:1
- Mate:37: 30 - Eccentric Rod 2:1 ↔ 31 - Lever:1
- Cylindrical:58: 32 - Eccentric Disk Rod:1 ↔ 30 - Eccentric Rod 2:2
- Mate:38: 32 - Eccentric Disk Rod:1 ↔ 30 - Eccentric Rod 2:2
- Cylindrical:59: 31 - Lever:1 ↔ 30 - Eccentric Rod 2:2
- Mate:39: 31 - Lever:1 ↔ 30 - Eccentric Rod 2:2
- Cylindrical:60: 04B - Guide Support 2:1 ↔ 31 - Lever:1
- Cylindrical:61: 06 - Cylinder:1 ↔ 22 - Valve Disc Hub:2
- Mate:40: 06 - Cylinder:1 ↔ 22 - Valve Disc Hub:2
- Cylindrical:62: 32 - Eccentric Disk Rod:1 ↔ 33 - Eccentric Swivel Screw:1
- Cylindrical:63: 22 - Valve Disc Hub:2 ↔ 24 - Valve Disc Spindle:1
- Flush:8: 22 - Valve Disc Hub:2 ↔ 24 - Valve Disc Spindle:1
- Mate:41: 24 - Valve Disc Spindle:1 ↔ 23 - Valve Disc:1
- Mate:42: 24 - Valve Disc Spindle:1 ↔ 23 - Valve Disc:1
- Cylindrical:64: 33 - Eccentric Swivel Screw:1 ↔ 23 - Valve Disc:1
- Flush:9: 24 - Valve Disc Spindle:1 ↔ 23 - Valve Disc:1
- Mate:43: 24 - Valve Disc Spindle:1 ↔ ANSI B18.2.4.2M M3x0.5:1
- Mate:44: 24 - Valve Disc Spindle:1 ↔ ANSI B18.2.4.2M M3x0.5:1
- Cylindrical:65: 12B VALVE BONNET:3 ↔ 27 - Valve Level:1
- Cylindrical:66: 12B VALVE BONNET:1 ↔ 27 - Valve Level:2
- Cylindrical:67: 12B VALVE BONNET:2 ↔ 27 - Valve Level:3
- Cylindrical:68: 12B VALVE BONNET:4 ↔ 27 - Valve Level:4
- Mate:45: 12B VALVE BONNET:3 ↔ 27 - Valve Level:1
- Mate:46: 12B VALVE BONNET:1 ↔ 27 - Valve Level:2
- Mate:47: 12B VALVE BONNET:2 ↔ 27 - Valve Level:3
- Mate:48: 12B VALVE BONNET:4 ↔ 27 - Valve Level:4
- Cylindrical:69: 08 CYLINDER REAR COVER:1 ↔ 11 CROSSHEAD GUIDE:1
- Cylindrical:70: 04A - Guide Support 1:1 ↔ 11 CROSSHEAD GUIDE:1
- Mate:49: 25 - Disc Arm 1:4 ↔ 25 - Disc Arm 2:1
- Mate:50: 25 - Disc Arm 1:4 ↔ 25 - Disc Arm 2:1
- Mate:51: 25 - Disc Arm 1:5 ↔ 25 - Disc Arm 2:1
- Mate:52: 25 - Disc Arm 1:3 ↔ 25 - Disc Arm 2:2
- Mate:53: 25 - Disc Arm 1:6 ↔ 25 - Disc Arm 2:2
- Mate:54: 25 - Disc Arm 1:2 ↔ 25 - Disc Arm 2:3
- Mate:55: 25 - Disc Arm 1:7 ↔ 25 - Disc Arm 2:3
- Mate:56: 25 - Disc Arm 1:1 ↔ 25 - Disc Arm 2:4
- Mate:57: 25 - Disc Arm 1:8 ↔ 25 - Disc Arm 2:4
- Cylindrical:71: 27 - Valve Level:1 ↔ 25 - Disc Arm 1:5
- Cylindrical:72: 27 - Valve Level:2 ↔ 25 - Disc Arm 1:8
- Cylindrical:73: 27 - Valve Level:4 ↔ 25 - Disc Arm 1:2
- Cylindrical:74: 27 - Valve Level:3 ↔ 25 - Disc Arm 1:6
- Mate:58: 27 - Valve Level:1 ↔ 25 - Disc Arm 1:4
- Mate:59: 27 - Valve Level:2 ↔ 25 - Disc Arm 1:8
- Mate:60: 27 - Valve Level:3 ↔ 25 - Disc Arm 1:6
- Mate:61: 27 - Valve Level:4 ↔ 25 - Disc Arm 1:2
- Cylindrical:75: 23 - Valve Disc:1 ↔ 25 - Disc Arm 1:4
- Cylindrical:76: 23 - Valve Disc:1 ↔ 25 - Disc Arm 1:1
- Cylindrical:77: 23 - Valve Disc:1 ↔ 25 - Disc Arm 1:7
- Cylindrical:78: 23 - Valve Disc:1 ↔ 25 - Disc Arm 1:3
- Mate:62: 26B - Valve spindle:1 ↔ 26A - Valve:1
- Cylindrical:79: 26B - Valve spindle:1 ↔ 26A - Valve:1
- Mate:63: 26B - Valve spindle:1 ↔ 26A - Valve:1
- [Mate]: 26B - Valve spindle:2 ↔ 26A - Valve:2
- [CylindricalJoint]: 26B - Valve spindle:2 ↔ 26A - Valve:2
- [Mate]: 26B - Valve spindle:2 ↔ 26A - Valve:2
- [Mate]: 26B - Valve spindle:3 ↔ 26A - Valve:3
- [CylindricalJoint]: 26B - Valve spindle:3 ↔ 26A - Valve:3
- [Mate]: 26B - Valve spindle:3 ↔ 26A - Valve:3
- [Mate]: 26B - Valve spindle:4 ↔ 26A - Valve:4
- [CylindricalJoint]: 26B - Valve spindle:4 ↔ 26A - Valve:4
- [Mate]: 26B - Valve spindle:4 ↔ 26A - Valve:4
- Cylindrical:83: 27 - Valve Level:4 ↔ 26B - Valve spindle:1
- Cylindrical:84: 27 - Valve Level:1 ↔ 26B - Valve spindle:2
- Cylindrical:85: 27 - Valve Level:2 ↔ 26B - Valve spindle:3
- Cylindrical:86: 27 - Valve Level:3 ↔ 26B - Valve spindle:4
- Cylindrical:87: 10a GLAND NUT:1 ↔ 10B - Gland Nut Seal:1
- Mate:70: 10a GLAND NUT:1 ↔ 10B - Gland Nut Seal:1
- Mate:71: 08 CYLINDER REAR COVER:1 ↔ 10B - Gland Nut Seal:1
- Cylindrical:88: 19 - Crosshead:1 ↔ 18 - Piston Rod:1
- Mate:72: 19 - Crosshead:1 ↔ 18 - Piston Rod:1
- Cylindrical:89: 21 - Piston Ring:1 ↔ 20 - Piston:1
- Mate:73 (1.5 mm): 21 - Piston Ring:1 ↔ 20 - Piston:1
- Cylindrical:90: 18 - Piston Rod:1 ↔ 20 - Piston:1
- Flush:10: 18 - Piston Rod:1 ↔ 20 - Piston:1
- Cylindrical:91: 11 CROSSHEAD GUIDE:1 ↔ 20 - Piston:1
- Mate:74: 08 CYLINDER REAR COVER:1 ↔ 11 CROSSHEAD GUIDE:1
- Mate:75: 16B2 - Con Head Big End:1 ↔ 16A - Con Rod:1
- Mate:76: 16C - Con Head Crosshead:1 ↔ 16A - Con Rod:1
- Cylindrical:92: 16C - Con Head Crosshead:1 ↔ 17B - Crosshead Pin2:1
- Mate:77: 16C - Con Head Crosshead:1 ↔ 17B - Crosshead Pin2:1
- Cylindrical:93: 19 - Crosshead:1 ↔ 17B - Crosshead Pin2:1
- Cylindrical:94: 16C - Con Head Crosshead:1 ↔ 16A - Con Rod:1
- Cylindrical:95: 16B2 - Con Head Big End:1 ↔ 16A - Con Rod:1
- Mate:78: 16C - Con Head Crosshead:1 ↔ 19 - Crosshead:1
- Cylindrical:96: Crankshaft:1 ↔ 16B2 - Con Head Big End:1
- Cylindrical:97: 16B2 - Con Head Big End:1 ↔ Crankpin:1
## Named parameters: d552_d548 = 0 mm, d553_d549 = -54.536721 deg, d554_d550 = 0.1 mm, d555_d551 = 0 mm, d556_d548 = 0 mm, d557_d549 = -54.536721 deg, d558_d550 = 0.1 mm, d559_d551 = 0 mm, d560_d548 = 0 mm, d561_d549 = -54.536721 deg, d562_d550 = 0.1 mm, d563_d551 = 0 mm
